# Autodesk Inventor assembly: FaceShield_Assembly
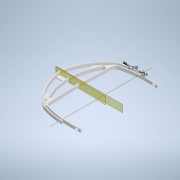
[picture p0: Inventor's stored thumbnail of the model, 180x180]
Saved by Autodesk Inventor 2020 (Build 240168000, 168)
## iProperties
Created: 2020-04-14
Part Number: FaceShield_Assembly
Document SubType Name: Assembly
Designer: maple
Author: maple
## Documents named in this file (3)
- C:\Nitro\Github\FaceShield\Ver 2\FaceShield_Assembly.iam
- C:\Nitro\Github\FaceShield\Ver 2\FaceShield_Part1.ipt
- C:\Nitro\Github\FaceShield\Ver 2\FaceShield_Part2.ipt
## Components (2 placed, 2 different names)
1. FaceShield_Part1:1 — Mate:1, Mate:2
2. FaceShield_Part2:1 — Mate:1, Mate:2
## Relationships (2: Mate 2)
- Mate:1: FaceShield_Part1:1 ↔ FaceShield_Part2:1
- Mate:2: FaceShield_Part1:1 ↔ FaceShield_Part2:1
